# Autodesk Inventor assembly: 13 in^3 drivetrain
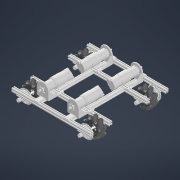
[picture p0: Inventor's stored thumbnail of the model, 180x180]
Saved by Autodesk Inventor 2022 (Build 260153000, 153)
## iProperties
Created: 2021-10-01
Part Number: 13 in^3 drivetrain
Document SubType Name: Assembly
Designer: izack
Author: izack
## Documents named in this file (13)
- D:\Robotics\ComputerAidedDesign\2021-22\FTC\#13822 Robovikes\Proof of Concept\13 in^3 drivetrain.iam
- D:\Robotics\ComputerAidedDesign\2021-22\FTC\#13822 Robovikes\Proof of Concept\13in^3 drivetrain parts\15mm Extrusion - 330.2mm - 90° Ends.ipt
- D:\Robotics\ComputerAidedDesign\2021-22\FTC\#13822 Robovikes\Proof of Concept\13in^3 drivetrain parts\15mm Bearing Pillow Block - 8 Pack.ipt
- D:\Robotics\ComputerAidedDesign\2021-22\FTC\#13822 Robovikes\Proof of Concept\13in^3 drivetrain parts\Through Bore Bearing - Long - 12 Pack.ipt
- D:\Robotics\ComputerAidedDesign\2021-22\FTC\#13822 Robovikes\Proof of Concept\13in^3 drivetrain parts\5mm x 100mm Hex Shaft - 4 Pack.ipt
- D:\Robotics\ComputerAidedDesign\2021-22\FTC\#13822 Robovikes\Proof of Concept\13in^3 drivetrain parts\Shaft Collars - 10 Pack.ipt
- D:\Robotics\ComputerAidedDesign\2021-22\FTC\#13822 Robovikes\Proof of Concept\13in^3 drivetrain parts\75mm Mecanum Wheel Set.iam
- D:\Robotics\ComputerAidedDesign\2021-22\FTC\#13822 Robovikes\Proof of Concept\13in^3 drivetrain parts\15mm Extrusion - 2.5in - 90° Ends.ipt
- D:\Robotics\ComputerAidedDesign\2021-22\FTC\#13822 Robovikes\Proof of Concept\13in^3 drivetrain parts\15mm Extrusion - 5.637 in - 90° Ends.ipt
- D:\Robotics\ComputerAidedDesign\2021-22\FTC\#13822 Robovikes\Proof of Concept\13in^3 drivetrain parts\5202 Series Yellow Jacket planetary Gear Motor Mount.ipt
- D:\Robotics\ComputerAidedDesign\2021-22\FTC\#13822 Robovikes\Proof of Concept\13in^3 drivetrain parts\5202 Series Yellow Jacket Planetary Gear Motor.ipt
- D:\Robotics\ComputerAidedDesign\2021-22\FTC\#13822 Robovikes\Proof of Concept\13in^3 drivetrain parts\26 Tooth #25 Sprocket - 4 Pack.ipt
- D:\Robotics\ComputerAidedDesign\2021-22\FTC\#13822 Robovikes\Proof of Concept\13in^3 drivetrain parts\10 Tooth #25 D-Shaft Sprocket - 4 Pack.ipt
## Components (58 placed, 12 different names)
1. 15mm Extrusion - 330.2mm - 90° Ends:1 — Flush:5, Mate:6, Flush:7, Flush:8, Flush:15, Mate:8, Mate:12, Mate:16, Mate:25, Mate:68, Mate:69, Mate:72, Flush:31, Flush:32, Flush:34, Mate:77
2. 15mm Extrusion - 330.2mm - 90° Ends:4 — Mate:6, Flush:7, Flush:9, Flush:14, Mate:9, Mate:13, Mate:17, Mate:24, Mate:62, Mate:63, Flush:22, Flush:23, Mate:70, Mate:71, Flush:24, Flush:25, Flush:30, Flush:33, Flush:35
3. 15mm Extrusion - 330.2mm - 90° Ends:5 — Mate:4, Flush:6, Flush:11, Flush:12, Mate:10, Mate:14, Mate:18, Mate:23, Mate:64, Mate:65, Mate:66, Mate:67, Flush:20, Flush:21, Mate:79, Flush:36, Flush:37, Flush:38, Flush:39, Mate:89, Flush:40
4. 15mm Extrusion - 330.2mm - 90° Ends:6 — Flush:5, Mate:4, Flush:6, Flush:13, Mate:11, Flush:10, Mate:15, Mate:19, Mate:22
5. 15mm Bearing Pillow Block - 8 Pack:1 — Flush:9, Mate:9, Mate:17, Rotational:2
6. 15mm Bearing Pillow Block - 8 Pack:2 — Flush:8, Mate:8, Mate:16, Rotational:1, Mate:100
7. 15mm Bearing Pillow Block - 8 Pack:3 — Flush:11, Mate:10, Mate:18, Rotational:3
8. 15mm Bearing Pillow Block - 8 Pack:4 — Flush:10, Mate:11, Mate:19, Rotational:4, Mate:94
9. 15mm Bearing Pillow Block - 8 Pack:5 — Flush:13, Mate:15, Rotational:5, Mate:22, Mate:97
10. 15mm Bearing Pillow Block - 8 Pack:6 — Flush:12, Mate:14, Rigid:2, Mate:23
11. 15mm Bearing Pillow Block - 8 Pack:7 — Flush:14, Mate:13, Rigid:1, Mate:24
12. 15mm Bearing Pillow Block - 8 Pack:8 — Flush:15, Mate:12, Rotational:6, Mate:25, Mate:103
13. Through Bore Bearing - Long - 12 Pack:1 — Rotational:1, Mate:26, Mate:44, Mate:45
14. Through Bore Bearing - Long - 12 Pack:2 — Rotational:3, Mate:27, Mate:28, Mate:29, Mate:46, Mate:47
15. Through Bore Bearing - Long - 12 Pack:3 — Rigid:1, Mate:34, Mate:35, Mate:40, Mate:41
16. Through Bore Bearing - Long - 12 Pack:4 — Rotational:6, Mate:36, Mate:37, Mate:38, Mate:39
17. Through Bore Bearing - Long - 12 Pack:5 — Rigid:2, Mate:33, Mate:42, Mate:43
18. Through Bore Bearing - Long - 12 Pack:6 — Rotational:5, Mate:31, Mate:32, Mate:48, Mate:49
19. Through Bore Bearing - Long - 12 Pack:7 — Rotational:4, Mate:30, Mate:50, Mate:51
20. Through Bore Bearing - Long - 12 Pack:8 — Rotational:2, Mate:20, Mate:21, Mate:52, Mate:53
21. 5mm x 100mm Hex Shaft - 4 Pack:1 — Mate:20, Mate:21, Mate:26, Flush:19, Mate:54, Mate:55, Mate:98, Mate:99
22. 5mm x 100mm Hex Shaft - 4 Pack:2 — Mate:27, Mate:28, Mate:29, Mate:30, Flush:18, Mate:60, Mate:61, Mate:90, Mate:91, Mate:92, Mate:93
23. 5mm x 100mm Hex Shaft - 4 Pack:3 — Mate:31, Mate:32, Mate:33, Flush:17, Mate:58, Mate:59, Mate:95, Mate:96
24. 5mm x 100mm Hex Shaft - 4 Pack:4 — Mate:34, Mate:35, Mate:36, Mate:37, Flush:16, Mate:56, Mate:57, Mate:101, Mate:102
25. Shaft Collars - 10 Pack:1 — Mate:50, Mate:51, Flush:18
26. Shaft Collars - 10 Pack:2 — Mate:52, Mate:53
27. Shaft Collars - 10 Pack:3 — Mate:38, Mate:39, Flush:16
28. Shaft Collars - 10 Pack:4 — Mate:40, Mate:41
29. Shaft Collars - 10 Pack:5 — Mate:48, Mate:49, Flush:17
30. Shaft Collars - 10 Pack:6 — Mate:46, Mate:47
31. Shaft Collars - 10 Pack:7 — Mate:44, Mate:45, Flush:19
32. Shaft Collars - 10 Pack:8 — Mate:42, Mate:43
33. 75mm Mecanum Wheel Set:1 [sub-assembly] — Mate:54, Mate:55, Mate:63
34. 75mm Mecanum Wheel Set:2 [sub-assembly] — Mate:60, Mate:61, Mate:65
35. 75mm Mecanum Wheel Set:3 [sub-assembly] — Mate:58, Mate:59, Mate:64
36. 75mm Mecanum Wheel Set:4 [sub-assembly] — Mate:56, Mate:57, Mate:62
37. 15mm Extrusion - 2.5in - 90° Ends:1 — Mate:66, Flush:21, Flush:27, Flush:42, Flush:43
38. 15mm Extrusion - 2.5in - 90° Ends:2 — Mate:67, Flush:20, Flush:28, Mate:78, Flush:41
39. 15mm Extrusion - 2.5in - 90° Ends:3 — Mate:68, Flush:22, Flush:26, Flush:32
40. 15mm Extrusion - 2.5in - 90° Ends:4 — Mate:69, Flush:23, Flush:29, Flush:33
41. 15mm Extrusion - 5.637 in - 90° Ends:1 — Mate:70, Flush:24, Flush:26, Flush:27, Mate:89, Flush:42, Flush:43
42. 15mm Extrusion - 5.637 in - 90° Ends:2 — Mate:71, Flush:25, Flush:28, Flush:29, Flush:40, Flush:41
43. 5202 Series Yellow Jacket planetary Gear Motor Mount:1 — Mate:72, Flush:30, Mate:74, Mate:75, Mate:76, Flush:31
44. 5202 Series Yellow Jacket Planetary Gear Motor:1 — Mate:74, Mate:75, Mate:76, Mate:106, Mate:109
45. 5202 Series Yellow Jacket planetary Gear Motor Mount:2 — Flush:34, Flush:35, Mate:77, Mate:80, Mate:83, Mate:84
46. 5202 Series Yellow Jacket planetary Gear Motor Mount:3 — Mate:78, Flush:37, Flush:39, Mate:81, Mate:85, Mate:86
47. 5202 Series Yellow Jacket planetary Gear Motor Mount:4 — Mate:79, Flush:36, Flush:38, Mate:82, Mate:87, Mate:88
48. 5202 Series Yellow Jacket Planetary Gear Motor:2 — Mate:82, Mate:87, Mate:88, Mate:108, Mate:110
49. 5202 Series Yellow Jacket Planetary Gear Motor:3 — Mate:81, Mate:85, Mate:86, Mate:107, Mate:111
50. 5202 Series Yellow Jacket Planetary Gear Motor:4 — Mate:80, Mate:83, Mate:84, Mate:104, Mate:105
51. 26 Tooth #25 Sprocket - 4 Pack:1 — Mate:90, Mate:91, Mate:92, Mate:93, Mate:94, Flush:45
52. 26 Tooth #25 Sprocket - 4 Pack:2 — Mate:95, Mate:96, Mate:97, Flush:46
53. 26 Tooth #25 Sprocket - 4 Pack:3 — Mate:98, Mate:99, Mate:100, Flush:44
54. 26 Tooth #25 Sprocket - 4 Pack:4 — Mate:101, Mate:102, Mate:103, Flush:47
55. 10 Tooth #25 D-Shaft Sprocket - 4 Pack:1 — Mate:104, Mate:105, Flush:44
56. 10 Tooth #25 D-Shaft Sprocket - 4 Pack:2 — Mate:107, Mate:111, Flush:45
57. 10 Tooth #25 D-Shaft Sprocket - 4 Pack:3 — Mate:106, Mate:109, Flush:47
58. 10 Tooth #25 D-Shaft Sprocket - 4 Pack:4 — Mate:108, Mate:110, Flush:46
## Relationships (156: Mate 105, Flush 43, RevoluteJoint 6, WeldJoint 2)
- Flush:5: 15mm Extrusion - 330.2mm - 90° Ends:1 ↔ 15mm Extrusion - 330.2mm - 90° Ends:6
- Mate:4 (63.5 mm): 15mm Extrusion - 330.2mm - 90° Ends:5 ↔ 15mm Extrusion - 330.2mm - 90° Ends:6
- Flush:6: 15mm Extrusion - 330.2mm - 90° Ends:5 ↔ 15mm Extrusion - 330.2mm - 90° Ends:6
- Mate:6 (63.5 mm): 15mm Extrusion - 330.2mm - 90° Ends:1 ↔ 15mm Extrusion - 330.2mm - 90° Ends:4
- Flush:7: 15mm Extrusion - 330.2mm - 90° Ends:1 ↔ 15mm Extrusion - 330.2mm - 90° Ends:4
- Flush:8: 15mm Extrusion - 330.2mm - 90° Ends:1 ↔ 15mm Bearing Pillow Block - 8 Pack:2
- Flush:9: 15mm Extrusion - 330.2mm - 90° Ends:4 ↔ 15mm Bearing Pillow Block - 8 Pack:1
- Flush:10: 15mm Extrusion - 330.2mm - 90° Ends:6 ↔ 15mm Bearing Pillow Block - 8 Pack:4
- Flush:11: 15mm Extrusion - 330.2mm - 90° Ends:5 ↔ 15mm Bearing Pillow Block - 8 Pack:3
- Flush:12: 15mm Extrusion - 330.2mm - 90° Ends:5 ↔ 15mm Bearing Pillow Block - 8 Pack:6
- Flush:13: 15mm Extrusion - 330.2mm - 90° Ends:6 ↔ 15mm Bearing Pillow Block - 8 Pack:5
- Flush:14: 15mm Extrusion - 330.2mm - 90° Ends:4 ↔ 15mm Bearing Pillow Block - 8 Pack:7
- Flush:15: 15mm Extrusion - 330.2mm - 90° Ends:1 ↔ 15mm Bearing Pillow Block - 8 Pack:8
- Mate:8: 15mm Extrusion - 330.2mm - 90° Ends:1 ↔ 15mm Bearing Pillow Block - 8 Pack:2
- Mate:9: 15mm Extrusion - 330.2mm - 90° Ends:4 ↔ 15mm Bearing Pillow Block - 8 Pack:1
- Mate:10: 15mm Extrusion - 330.2mm - 90° Ends:5 ↔ 15mm Bearing Pillow Block - 8 Pack:3
- Mate:11: 15mm Extrusion - 330.2mm - 90° Ends:6 ↔ 15mm Bearing Pillow Block - 8 Pack:4
- Mate:12: 15mm Extrusion - 330.2mm - 90° Ends:1 ↔ 15mm Bearing Pillow Block - 8 Pack:8
- Mate:13: 15mm Extrusion - 330.2mm - 90° Ends:4 ↔ 15mm Bearing Pillow Block - 8 Pack:7
- Mate:14: 15mm Extrusion - 330.2mm - 90° Ends:5 ↔ 15mm Bearing Pillow Block - 8 Pack:6
- Mate:15: 15mm Extrusion - 330.2mm - 90° Ends:6 ↔ 15mm Bearing Pillow Block - 8 Pack:5
- Mate:16 (-19.05 mm): 15mm Extrusion - 330.2mm - 90° Ends:1 ↔ 15mm Bearing Pillow Block - 8 Pack:2
- Mate:17 (-19.05 mm): 15mm Extrusion - 330.2mm - 90° Ends:4 ↔ 15mm Bearing Pillow Block - 8 Pack:1
- Mate:18 (-19.05 mm): 15mm Extrusion - 330.2mm - 90° Ends:5 ↔ 15mm Bearing Pillow Block - 8 Pack:3
- Mate:19 (-19.05 mm): 15mm Extrusion - 330.2mm - 90° Ends:6 ↔ 15mm Bearing Pillow Block - 8 Pack:4
- Rotational:1 [RevoluteJoint]: 15mm Bearing Pillow Block - 8 Pack:2 ↔ Through Bore Bearing - Long - 12 Pack:1
- Rotational:2 [RevoluteJoint]: 15mm Bearing Pillow Block - 8 Pack:1 ↔ Through Bore Bearing - Long - 12 Pack:8
- Rotational:3 [RevoluteJoint]: 15mm Bearing Pillow Block - 8 Pack:3 ↔ Through Bore Bearing - Long - 12 Pack:2
- Rotational:4 [RevoluteJoint]: 15mm Bearing Pillow Block - 8 Pack:4 ↔ Through Bore Bearing - Long - 12 Pack:7
- Rotational:5 [RevoluteJoint]: 15mm Bearing Pillow Block - 8 Pack:5 ↔ Through Bore Bearing - Long - 12 Pack:6
- Rigid:1 [WeldJoint]: 15mm Bearing Pillow Block - 8 Pack:7 ↔ Through Bore Bearing - Long - 12 Pack:3
- Rigid:2 [WeldJoint]: 15mm Bearing Pillow Block - 8 Pack:6 ↔ Through Bore Bearing - Long - 12 Pack:5
- Rotational:6 [RevoluteJoint]: 15mm Bearing Pillow Block - 8 Pack:8 ↔ Through Bore Bearing - Long - 12 Pack:4
- Mate:20: Through Bore Bearing - Long - 12 Pack:8 ↔ 5mm x 100mm Hex Shaft - 4 Pack:1
- Mate:21: Through Bore Bearing - Long - 12 Pack:8 ↔ 5mm x 100mm Hex Shaft - 4 Pack:1
- Mate:22 (-19.05 mm): 15mm Extrusion - 330.2mm - 90° Ends:6 ↔ 15mm Bearing Pillow Block - 8 Pack:5
- Mate:23 (-19.05 mm): 15mm Extrusion - 330.2mm - 90° Ends:5 ↔ 15mm Bearing Pillow Block - 8 Pack:6
- Mate:24 (-19.05 mm): 15mm Extrusion - 330.2mm - 90° Ends:4 ↔ 15mm Bearing Pillow Block - 8 Pack:7
- Mate:25 (-19.05 mm): 15mm Extrusion - 330.2mm - 90° Ends:1 ↔ 15mm Bearing Pillow Block - 8 Pack:8
- Mate:26: Through Bore Bearing - Long - 12 Pack:1 ↔ 5mm x 100mm Hex Shaft - 4 Pack:1
- Mate:27: Through Bore Bearing - Long - 12 Pack:2 ↔ 5mm x 100mm Hex Shaft - 4 Pack:2
- Mate:28: Through Bore Bearing - Long - 12 Pack:2 ↔ 5mm x 100mm Hex Shaft - 4 Pack:2
- Mate:29: Through Bore Bearing - Long - 12 Pack:2 ↔ 5mm x 100mm Hex Shaft - 4 Pack:2
- Mate:30: Through Bore Bearing - Long - 12 Pack:7 ↔ 5mm x 100mm Hex Shaft - 4 Pack:2
- Mate:31: Through Bore Bearing - Long - 12 Pack:6 ↔ 5mm x 100mm Hex Shaft - 4 Pack:3
- Mate:32: Through Bore Bearing - Long - 12 Pack:6 ↔ 5mm x 100mm Hex Shaft - 4 Pack:3
- Mate:33: Through Bore Bearing - Long - 12 Pack:5 ↔ 5mm x 100mm Hex Shaft - 4 Pack:3
- Mate:34: Through Bore Bearing - Long - 12 Pack:3 ↔ 5mm x 100mm Hex Shaft - 4 Pack:4
- Mate:35: Through Bore Bearing - Long - 12 Pack:3 ↔ 5mm x 100mm Hex Shaft - 4 Pack:4
- Mate:36: Through Bore Bearing - Long - 12 Pack:4 ↔ 5mm x 100mm Hex Shaft - 4 Pack:4
- Mate:37: Through Bore Bearing - Long - 12 Pack:4 ↔ 5mm x 100mm Hex Shaft - 4 Pack:4
- Mate:38: Through Bore Bearing - Long - 12 Pack:4 ↔ Shaft Collars - 10 Pack:3
- Mate:39: Through Bore Bearing - Long - 12 Pack:4 ↔ Shaft Collars - 10 Pack:3
- Flush:16: 5mm x 100mm Hex Shaft - 4 Pack:4 ↔ Shaft Collars - 10 Pack:3
- Mate:40: Through Bore Bearing - Long - 12 Pack:3 ↔ Shaft Collars - 10 Pack:4
- Mate:41: Through Bore Bearing - Long - 12 Pack:3 ↔ Shaft Collars - 10 Pack:4
- Mate:42: Through Bore Bearing - Long - 12 Pack:5 ↔ Shaft Collars - 10 Pack:8
- Mate:43: Through Bore Bearing - Long - 12 Pack:5 ↔ Shaft Collars - 10 Pack:8
- Mate:44: Through Bore Bearing - Long - 12 Pack:1 ↔ Shaft Collars - 10 Pack:7
- Mate:45: Through Bore Bearing - Long - 12 Pack:1 ↔ Shaft Collars - 10 Pack:7
- Mate:46: Through Bore Bearing - Long - 12 Pack:2 ↔ Shaft Collars - 10 Pack:6
- Mate:47: Through Bore Bearing - Long - 12 Pack:2 ↔ Shaft Collars - 10 Pack:6
- Mate:48: Through Bore Bearing - Long - 12 Pack:6 ↔ Shaft Collars - 10 Pack:5
- Mate:49: Through Bore Bearing - Long - 12 Pack:6 ↔ Shaft Collars - 10 Pack:5
- Mate:50: Through Bore Bearing - Long - 12 Pack:7 ↔ Shaft Collars - 10 Pack:1
- Mate:51: Through Bore Bearing - Long - 12 Pack:7 ↔ Shaft Collars - 10 Pack:1
- Mate:52: Through Bore Bearing - Long - 12 Pack:8 ↔ Shaft Collars - 10 Pack:2
- Mate:53: Through Bore Bearing - Long - 12 Pack:8 ↔ Shaft Collars - 10 Pack:2
- Flush:17: 5mm x 100mm Hex Shaft - 4 Pack:3 ↔ Shaft Collars - 10 Pack:5
- Flush:18: 5mm x 100mm Hex Shaft - 4 Pack:2 ↔ Shaft Collars - 10 Pack:1
- Flush:19: 5mm x 100mm Hex Shaft - 4 Pack:1 ↔ Shaft Collars - 10 Pack:7
- Mate:54: 5mm x 100mm Hex Shaft - 4 Pack:1 ↔ 75mm Mecanum Wheel Set:1
- Mate:55: 5mm x 100mm Hex Shaft - 4 Pack:1 ↔ 75mm Mecanum Wheel Set:1
- Mate:56: 5mm x 100mm Hex Shaft - 4 Pack:4 ↔ 75mm Mecanum Wheel Set:4
- Mate:57: 5mm x 100mm Hex Shaft - 4 Pack:4 ↔ 75mm Mecanum Wheel Set:4
- Mate:58: 5mm x 100mm Hex Shaft - 4 Pack:3 ↔ 75mm Mecanum Wheel Set:3
- Mate:59: 5mm x 100mm Hex Shaft - 4 Pack:3 ↔ 75mm Mecanum Wheel Set:3
- Mate:60: 5mm x 100mm Hex Shaft - 4 Pack:2 ↔ 75mm Mecanum Wheel Set:2
- Mate:61: 5mm x 100mm Hex Shaft - 4 Pack:2 ↔ 75mm Mecanum Wheel Set:2
- Mate:62 (16.51 mm): 15mm Extrusion - 330.2mm - 90° Ends:4 ↔ 75mm Mecanum Wheel Set:4
- Mate:63 (16.51 mm): 15mm Extrusion - 330.2mm - 90° Ends:4 ↔ 75mm Mecanum Wheel Set:1
- Mate:64 (21.082 mm): 15mm Extrusion - 330.2mm - 90° Ends:5 ↔ 75mm Mecanum Wheel Set:3
- Mate:65 (21.082 mm): 15mm Extrusion - 330.2mm - 90° Ends:5 ↔ 75mm Mecanum Wheel Set:2
- Mate:66: 15mm Extrusion - 330.2mm - 90° Ends:5 ↔ 15mm Extrusion - 2.5in - 90° Ends:1
- Mate:67: 15mm Extrusion - 330.2mm - 90° Ends:5 ↔ 15mm Extrusion - 2.5in - 90° Ends:2
- Flush:20: 15mm Extrusion - 330.2mm - 90° Ends:5 ↔ 15mm Extrusion - 2.5in - 90° Ends:2
- Flush:21: 15mm Extrusion - 330.2mm - 90° Ends:5 ↔ 15mm Extrusion - 2.5in - 90° Ends:1
- Mate:68: 15mm Extrusion - 330.2mm - 90° Ends:1 ↔ 15mm Extrusion - 2.5in - 90° Ends:3
- Mate:69: 15mm Extrusion - 330.2mm - 90° Ends:1 ↔ 15mm Extrusion - 2.5in - 90° Ends:4
- Flush:22: 15mm Extrusion - 330.2mm - 90° Ends:4 ↔ 15mm Extrusion - 2.5in - 90° Ends:3
- Flush:23: 15mm Extrusion - 330.2mm - 90° Ends:4 ↔ 15mm Extrusion - 2.5in - 90° Ends:4
- Mate:70: 15mm Extrusion - 330.2mm - 90° Ends:4 ↔ 15mm Extrusion - 5.637 in - 90° Ends:1
- Mate:71: 15mm Extrusion - 330.2mm - 90° Ends:4 ↔ 15mm Extrusion - 5.637 in - 90° Ends:2
- Flush:24: 15mm Extrusion - 330.2mm - 90° Ends:4 ↔ 15mm Extrusion - 5.637 in - 90° Ends:1
- Flush:25: 15mm Extrusion - 330.2mm - 90° Ends:4 ↔ 15mm Extrusion - 5.637 in - 90° Ends:2
- Flush:26: 15mm Extrusion - 2.5in - 90° Ends:3 ↔ 15mm Extrusion - 5.637 in - 90° Ends:1
- Flush:27: 15mm Extrusion - 2.5in - 90° Ends:1 ↔ 15mm Extrusion - 5.637 in - 90° Ends:1
- Flush:28: 15mm Extrusion - 2.5in - 90° Ends:2 ↔ 15mm Extrusion - 5.637 in - 90° Ends:2
- Flush:29: 15mm Extrusion - 2.5in - 90° Ends:4 ↔ 15mm Extrusion - 5.637 in - 90° Ends:2
- Mate:72: 15mm Extrusion - 330.2mm - 90° Ends:1 ↔ 5202 Series Yellow Jacket planetary Gear Motor Mount:1
- Flush:30: 15mm Extrusion - 330.2mm - 90° Ends:4 ↔ 5202 Series Yellow Jacket planetary Gear Motor Mount:1
- Mate:74: 5202 Series Yellow Jacket planetary Gear Motor Mount:1 ↔ 5202 Series Yellow Jacket Planetary Gear Motor:1
- Mate:75: 5202 Series Yellow Jacket planetary Gear Motor Mount:1 ↔ 5202 Series Yellow Jacket Planetary Gear Motor:1
- Mate:76: 5202 Series Yellow Jacket planetary Gear Motor Mount:1 ↔ 5202 Series Yellow Jacket Planetary Gear Motor:1
- Flush:31 (76.2 mm): 15mm Extrusion - 330.2mm - 90° Ends:1 ↔ 5202 Series Yellow Jacket planetary Gear Motor Mount:1
- Flush:32 (93.0148 mm): 15mm Extrusion - 330.2mm - 90° Ends:1 ↔ 15mm Extrusion - 2.5in - 90° Ends:3
- Flush:33 (93.0148 mm): 15mm Extrusion - 330.2mm - 90° Ends:4 ↔ 15mm Extrusion - 2.5in - 90° Ends:4
- Flush:34 (76.2 mm): 15mm Extrusion - 330.2mm - 90° Ends:1 ↔ 5202 Series Yellow Jacket planetary Gear Motor Mount:2
- Flush:35: 15mm Extrusion - 330.2mm - 90° Ends:4 ↔ 5202 Series Yellow Jacket planetary Gear Motor Mount:2
- Mate:77: 15mm Extrusion - 330.2mm - 90° Ends:1 ↔ 5202 Series Yellow Jacket planetary Gear Motor Mount:2
- Mate:78: 15mm Extrusion - 2.5in - 90° Ends:2 ↔ 5202 Series Yellow Jacket planetary Gear Motor Mount:3
- Mate:79: 15mm Extrusion - 330.2mm - 90° Ends:5 ↔ 5202 Series Yellow Jacket planetary Gear Motor Mount:4
- Flush:36: 15mm Extrusion - 330.2mm - 90° Ends:5 ↔ 5202 Series Yellow Jacket planetary Gear Motor Mount:4
- Flush:37: 15mm Extrusion - 330.2mm - 90° Ends:5 ↔ 5202 Series Yellow Jacket planetary Gear Motor Mount:3
- Flush:38 (76.2 mm): 15mm Extrusion - 330.2mm - 90° Ends:5 ↔ 5202 Series Yellow Jacket planetary Gear Motor Mount:4
- Flush:39 (76.2 mm): 15mm Extrusion - 330.2mm - 90° Ends:5 ↔ 5202 Series Yellow Jacket planetary Gear Motor Mount:3
- Mate:80: 5202 Series Yellow Jacket planetary Gear Motor Mount:2 ↔ 5202 Series Yellow Jacket Planetary Gear Motor:4
- Mate:81: 5202 Series Yellow Jacket planetary Gear Motor Mount:3 ↔ 5202 Series Yellow Jacket Planetary Gear Motor:3
- Mate:82: 5202 Series Yellow Jacket planetary Gear Motor Mount:4 ↔ 5202 Series Yellow Jacket Planetary Gear Motor:2
- Mate:83: 5202 Series Yellow Jacket planetary Gear Motor Mount:2 ↔ 5202 Series Yellow Jacket Planetary Gear Motor:4
- Mate:84: 5202 Series Yellow Jacket planetary Gear Motor Mount:2 ↔ 5202 Series Yellow Jacket Planetary Gear Motor:4
- Mate:85: 5202 Series Yellow Jacket planetary Gear Motor Mount:3 ↔ 5202 Series Yellow Jacket Planetary Gear Motor:3
- Mate:86: 5202 Series Yellow Jacket planetary Gear Motor Mount:3 ↔ 5202 Series Yellow Jacket Planetary Gear Motor:3
- Mate:87: 5202 Series Yellow Jacket planetary Gear Motor Mount:4 ↔ 5202 Series Yellow Jacket Planetary Gear Motor:2
- Mate:88: 5202 Series Yellow Jacket planetary Gear Motor Mount:4 ↔ 5202 Series Yellow Jacket Planetary Gear Motor:2
- Mate:89: 15mm Extrusion - 330.2mm - 90° Ends:5 ↔ 15mm Extrusion - 5.637 in - 90° Ends:1
- Flush:40: 15mm Extrusion - 330.2mm - 90° Ends:5 ↔ 15mm Extrusion - 5.637 in - 90° Ends:2
- Flush:41: 15mm Extrusion - 2.5in - 90° Ends:2 ↔ 15mm Extrusion - 5.637 in - 90° Ends:2
- Flush:42: 15mm Extrusion - 2.5in - 90° Ends:1 ↔ 15mm Extrusion - 5.637 in - 90° Ends:1
- Flush:43: 15mm Extrusion - 2.5in - 90° Ends:1 ↔ 15mm Extrusion - 5.637 in - 90° Ends:1
- Mate:90: 5mm x 100mm Hex Shaft - 4 Pack:2 ↔ 26 Tooth #25 Sprocket - 4 Pack:1
- Mate:91: 5mm x 100mm Hex Shaft - 4 Pack:2 ↔ 26 Tooth #25 Sprocket - 4 Pack:1
- Mate:92: 5mm x 100mm Hex Shaft - 4 Pack:2 ↔ 26 Tooth #25 Sprocket - 4 Pack:1
- Mate:93: 5mm x 100mm Hex Shaft - 4 Pack:2 ↔ 26 Tooth #25 Sprocket - 4 Pack:1
- Mate:94 (2.54 mm): 15mm Bearing Pillow Block - 8 Pack:4 ↔ 26 Tooth #25 Sprocket - 4 Pack:1
- Mate:95: 5mm x 100mm Hex Shaft - 4 Pack:3 ↔ 26 Tooth #25 Sprocket - 4 Pack:2
- Mate:96: 5mm x 100mm Hex Shaft - 4 Pack:3 ↔ 26 Tooth #25 Sprocket - 4 Pack:2
- Mate:97 (2.54 mm): 15mm Bearing Pillow Block - 8 Pack:5 ↔ 26 Tooth #25 Sprocket - 4 Pack:2
- Mate:98: 5mm x 100mm Hex Shaft - 4 Pack:1 ↔ 26 Tooth #25 Sprocket - 4 Pack:3
- Mate:99: 5mm x 100mm Hex Shaft - 4 Pack:1 ↔ 26 Tooth #25 Sprocket - 4 Pack:3
- Mate:100 (2.54 mm): 15mm Bearing Pillow Block - 8 Pack:2 ↔ 26 Tooth #25 Sprocket - 4 Pack:3
- Mate:101: 5mm x 100mm Hex Shaft - 4 Pack:4 ↔ 26 Tooth #25 Sprocket - 4 Pack:4
- Mate:102: 5mm x 100mm Hex Shaft - 4 Pack:4 ↔ 26 Tooth #25 Sprocket - 4 Pack:4
- Mate:103 (2.54 mm): 15mm Bearing Pillow Block - 8 Pack:8 ↔ 26 Tooth #25 Sprocket - 4 Pack:4
- Mate:104: 5202 Series Yellow Jacket Planetary Gear Motor:4 ↔ 10 Tooth #25 D-Shaft Sprocket - 4 Pack:1
- Mate:105: 5202 Series Yellow Jacket Planetary Gear Motor:4 ↔ 10 Tooth #25 D-Shaft Sprocket - 4 Pack:1
- Flush:44: 26 Tooth #25 Sprocket - 4 Pack:3 ↔ 10 Tooth #25 D-Shaft Sprocket - 4 Pack:1
- Mate:106: 5202 Series Yellow Jacket Planetary Gear Motor:1 ↔ 10 Tooth #25 D-Shaft Sprocket - 4 Pack:3
- Mate:107: 5202 Series Yellow Jacket Planetary Gear Motor:3 ↔ 10 Tooth #25 D-Shaft Sprocket - 4 Pack:2
- Mate:108: 5202 Series Yellow Jacket Planetary Gear Motor:2 ↔ 10 Tooth #25 D-Shaft Sprocket - 4 Pack:4
- Mate:109: 5202 Series Yellow Jacket Planetary Gear Motor:1 ↔ 10 Tooth #25 D-Shaft Sprocket - 4 Pack:3
- Mate:110: 5202 Series Yellow Jacket Planetary Gear Motor:2 ↔ 10 Tooth #25 D-Shaft Sprocket - 4 Pack:4
- Mate:111: 5202 Series Yellow Jacket Planetary Gear Motor:3 ↔ 10 Tooth #25 D-Shaft Sprocket - 4 Pack:2
- Flush:45: 26 Tooth #25 Sprocket - 4 Pack:1 ↔ 10 Tooth #25 D-Shaft Sprocket - 4 Pack:2
- Flush:46: 26 Tooth #25 Sprocket - 4 Pack:2 ↔ 10 Tooth #25 D-Shaft Sprocket - 4 Pack:4
- Flush:47: 26 Tooth #25 Sprocket - 4 Pack:4 ↔ 10 Tooth #25 D-Shaft Sprocket - 4 Pack:3
